# Autodesk Inventor assembly: SPE1V1 Estructura
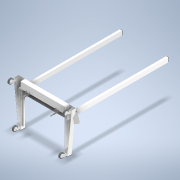
[picture p0: Inventor's stored thumbnail of the model, 180x180]
Saved by Autodesk Inventor 2021.2 (Build 252289000, 289)
## iProperties
Created: 2026-06-02
Part Number: SPE1V1 Estructura
Document SubType Name: Assembly
Designer: nelso
Author: nelso
## Documents named in this file (18)
- C:\Users\nelso\Desktop\Soporte-Paciente-Espinografia\Workspace\SPE1V1 Estructura.iam
- C:\Users\nelso\Desktop\Soporte-Paciente-Espinografia\Workspace\SP22V1 Tubo 40x80x1825mm.ipt
- C:\Users\nelso\Desktop\Soporte-Paciente-Espinografia\Workspace\SP21V1 Tubo 40x80x100mm.ipt
- C:\Users\nelso\Desktop\Soporte-Paciente-Espinografia\Workspace\SP23V1 Cobertora Derecha.ipt
- C:\Users\nelso\Desktop\Soporte-Paciente-Espinografia\Workspace\SP24V1 Cobertora Izquierda.ipt
- C:\Users\nelso\Desktop\Soporte-Paciente-Espinografia\Workspace\SP20V1 Tubo 80x120x790mm.ipt
- C:\Users\nelso\Desktop\Soporte-Paciente-Espinografia\Workspace\SP19V1 Tapacanto Delantero.ipt
- C:\Users\nelso\Desktop\Soporte-Paciente-Espinografia\Workspace\SP18V1 Tapacanto Superior.ipt
- C:\Users\nelso\Desktop\Soporte-Paciente-Espinografia\Workspace\RFPLUS8PO300.ipt
- C:\Users\nelso\Desktop\Soporte-Paciente-Espinografia\Workspace\SP17V1 Varilla Pedal.ipt
- C:\Users\nelso\Desktop\Soporte-Paciente-Espinografia\Workspace\SP16V1 Buje Pedal.ipt
- C:\Users\nelso\Desktop\Soporte-Paciente-Espinografia\Workspace\SP15V1 Pedal Izquierdo.ipt
- C:\Users\nelso\Desktop\Soporte-Paciente-Espinografia\Workspace\SPE3V1 Freno.iam
- C:\Users\nelso\Desktop\Soporte-Paciente-Espinografia\Workspace\SP14V1 Pedal Derecho.ipt
- C:\Users\nelso\Desktop\Soporte-Paciente-Espinografia\Workspace\5100B-HG-RU.ipt
- C:\Users\nelso\Desktop\Soporte-Paciente-Espinografia\Workspace\SP33V1 Tope Base.ipt
- C:\Users\nelso\Desktop\Soporte-Paciente-Espinografia\Workspace\SP38V1 Cobertor Freno.ipt
- C:\Users\nelso\Desktop\Soporte-Paciente-Espinografia\Workspace\SP43V1 Tubo 40x80x1825mm.ipt
## Components (42 placed, 17 different names)
1. SP43V1 Tubo 40x80x1825mm:1 — Nivelación:17, Coincidencia:54, Coincidencia:55, Coincidencia:68, Nivelación:67, Coincidencia:71, Flush:75, Flush:76, Flush:77, Flush:78, Flush:79, Mate:84, Mate:85, Mate:86, Mate:87, Mate:88, Mate:107, Flush:101
2. SP18V1 Tapacanto Superior:1 — Coincidencia:68, Nivelación:67, Coincidencia:71
3. SP22V1 Tubo 40x80x1825mm:2 — Mate:179, Mate:180, Flush:120, Mate:181, Mate:182, Mate:183, Mate:184, Mate:185, Mate:186, Mate:187, Flush:121, Flush:122, Flush:123, Flush:124, Flush:125, Flush:126
4. SP18V1 Tapacanto Superior:2 — Mate:181
5. SP21V1 Tubo 40x80x100mm:1 — Nivelación:14, Coincidencia:24, Coincidencia:42, Coincidencia:60, Coincidencia:62, Coincidencia:63, Mate:156, Mate:157
6. SP19V1 Tapacanto Delantero:1 — Coincidencia:60, Coincidencia:62, Coincidencia:63
7. SP21V1 Tubo 40x80x100mm:2 — Coincidencia:37, Coincidencia:38, Coincidencia:66, Mate:154, Mate:155
8. SP21V1 Tubo 40x80x100mm:3 — Coincidencia:50, Coincidencia:51, Coincidencia:65, Mate:158, Mate:159
9. SP21V1 Tubo 40x80x100mm:4 — Mate:150, Mate:151, Mate:160, Mate:161
10. SP19V1 Tapacanto Delantero:2 — Mate:152
11. SP23V1 Cobertora Derecha:1 — Nivelación:14, Coincidencia:24, Nivelación:17, Coincidencia:37, Coincidencia:38, Nivelación:18, Coincidencia:42, Nivelación:26, Coincidencia:55, Nivelación:27, Coincidencia:66, Flush:97, Flush:98, Mate:96, Mate:97, Flush:105, Mate:126, Mate:131, Mate:162, Mate:174, Flush:118
12. SP24V1 Cobertora Izquierda:1 — Nivelación:18, Coincidencia:50, Coincidencia:51, Nivelación:24, Coincidencia:53, Nivelación:28, Coincidencia:65, Flush:95, Flush:96, Mate:94, Mate:95, Flush:104, Mate:127, Mate:150, Mate:151, Mate:152, Mate:180, Flush:120
13. SP20V1 Tubo 80x120x790mm:1 — Nivelación:24, Nivelación:25, Coincidencia:54, Nivelación:27, Nivelación:28, Mate:110, Mate:111, Mate:124, Flush:119, Mate:177, Mate:179
14. RFPLUS8PO300:1 — Mate:107, Flush:101
15. RFPLUS8PO300:2 — Flush:75, Mate:88
16. RFPLUS8PO300:3 — Flush:76, Mate:87
17. RFPLUS8PO300:4 — Flush:77, Mate:86
18. RFPLUS8PO300:5 — Flush:78, Mate:84
19. RFPLUS8PO300:6 — Flush:79, Mate:85
20. RFPLUS8PO300:13 — Flush:95, Mate:94
21. RFPLUS8PO300:14 — Flush:96, Mate:95
22. RFPLUS8PO300:15 — Flush:97, Mate:97
23. RFPLUS8PO300:16 — Flush:98, Mate:96
24. SP17V1 Varilla Pedal:1 — Flush:102, Mate:117, Mate:118, Mate:119, Mate:120, Mate:121, Mate:125, Mate:128, Mate:129, Mate:130, Mate:132, Mate:133, Mate:134, Flush:106, Flush:107
25. SP16V1 Buje Pedal:1 — Mate:116, Flush:105, Mate:131
26. SP16V1 Buje Pedal:2 — Mate:116, Mate:125, Flush:104
27. SP14V1 Pedal Derecho:1 — Mate:128, Mate:129, Mate:130, Mate:132, Flush:107
28. SP15V1 Pedal Izquierdo:1 — Mate:120, Mate:121, Flush:106
29. SPE3V1 Freno:1 [sub-assembly] — Mate:110, Flush:103, Mate:117, Mate:118, Mate:119, Mate:124, Mate:127
30. SPE3V1 Freno:2 [sub-assembly] — Mate:111, Flush:103, Mate:126, Mate:133, Mate:134
31. RFPLUS8PO300:17 — Mate:187, Flush:121
32. RFPLUS8PO300:18 — Mate:186, Flush:122
33. RFPLUS8PO300:19 — Mate:185, Flush:123
34. RFPLUS8PO300:20 — Mate:184, Flush:124
35. RFPLUS8PO300:21 — Mate:182, Flush:125
36. RFPLUS8PO300:22 — Mate:183, Flush:126
37. 5100B-HG-RU:1 — Mate:154, Mate:155, Tangent:1
38. 5100B-HG-RU:2 — Mate:156, Mate:157
39. 5100B-HG-RU:3 — Mate:160, Mate:161
40. 5100B-HG-RU:4 — Mate:158, Mate:159
41. SP33V1 Tope Base:1 — Mate:174, Flush:118, Mate:178
42. SP38V1 Cobertor Freno:1 — Mate:176, Flush:119, Mate:177, Mate:178
## Relationships (110: Mate 74, Flush 35, Tangent 1)
- Nivelación:14 [Flush]: SP21V1 Tubo 40x80x100mm:1 ↔ SP23V1 Cobertora Derecha:1
- Coincidencia:24 [Mate] (0.5 mm): SP21V1 Tubo 40x80x100mm:1 ↔ SP23V1 Cobertora Derecha:1
- Nivelación:17 [Flush]: SP43V1 Tubo 40x80x1825mm:1 ↔ SP23V1 Cobertora Derecha:1
- Coincidencia:37 [Mate]: SP21V1 Tubo 40x80x100mm:2 ↔ SP23V1 Cobertora Derecha:1
- Coincidencia:38 [Mate]: SP21V1 Tubo 40x80x100mm:2 ↔ SP23V1 Cobertora Derecha:1
- Nivelación:18 [Flush]: SP23V1 Cobertora Derecha:1 ↔ SP24V1 Cobertora Izquierda:1
- Coincidencia:42 [Mate]: SP21V1 Tubo 40x80x100mm:1 ↔ SP23V1 Cobertora Derecha:1
- Coincidencia:50 [Mate]: SP21V1 Tubo 40x80x100mm:3 ↔ SP24V1 Cobertora Izquierda:1
- Coincidencia:51 [Mate]: SP21V1 Tubo 40x80x100mm:3 ↔ SP24V1 Cobertora Izquierda:1
- Nivelación:24 [Flush]: SP24V1 Cobertora Izquierda:1 ↔ SP20V1 Tubo 80x120x790mm:1
- Nivelación:25 [Flush]: SP20V1 Tubo 80x120x790mm:1
- Coincidencia:53 [Mate] (395 mm): SP24V1 Cobertora Izquierda:1
- Nivelación:26 [Flush] (395 mm): SP23V1 Cobertora Derecha:1
- Coincidencia:54 [Mate]: SP43V1 Tubo 40x80x1825mm:1 ↔ SP20V1 Tubo 80x120x790mm:1
- Coincidencia:55 [Mate]: SP43V1 Tubo 40x80x1825mm:1 ↔ SP23V1 Cobertora Derecha:1
- Nivelación:27 [Flush]: SP23V1 Cobertora Derecha:1 ↔ SP20V1 Tubo 80x120x790mm:1
- Nivelación:28 [Flush]: SP24V1 Cobertora Izquierda:1 ↔ SP20V1 Tubo 80x120x790mm:1
- Coincidencia:60 [Mate]: SP21V1 Tubo 40x80x100mm:1 ↔ SP19V1 Tapacanto Delantero:1
- Coincidencia:62 [Mate]: SP21V1 Tubo 40x80x100mm:1 ↔ SP19V1 Tapacanto Delantero:1
- Coincidencia:63 [Mate]: SP21V1 Tubo 40x80x100mm:1 ↔ SP19V1 Tapacanto Delantero:1
- Coincidencia:65 [Mate]: SP21V1 Tubo 40x80x100mm:3 ↔ SP24V1 Cobertora Izquierda:1
- Coincidencia:66 [Mate]: SP21V1 Tubo 40x80x100mm:2 ↔ SP23V1 Cobertora Derecha:1
- Coincidencia:68 [Mate]: SP43V1 Tubo 40x80x1825mm:1 ↔ SP18V1 Tapacanto Superior:1
- Nivelación:67 [Flush]: SP43V1 Tubo 40x80x1825mm:1 ↔ SP18V1 Tapacanto Superior:1
- Coincidencia:71 [Mate]: SP43V1 Tubo 40x80x1825mm:1 ↔ SP18V1 Tapacanto Superior:1
- Flush:75: SP43V1 Tubo 40x80x1825mm:1 ↔ RFPLUS8PO300:2
- Flush:76: SP43V1 Tubo 40x80x1825mm:1 ↔ RFPLUS8PO300:3
- Flush:77: SP43V1 Tubo 40x80x1825mm:1 ↔ RFPLUS8PO300:4
- Flush:78: SP43V1 Tubo 40x80x1825mm:1 ↔ RFPLUS8PO300:5
- Flush:79: SP43V1 Tubo 40x80x1825mm:1 ↔ RFPLUS8PO300:6
- Mate:84: SP43V1 Tubo 40x80x1825mm:1 ↔ RFPLUS8PO300:5
- Mate:85: SP43V1 Tubo 40x80x1825mm:1 ↔ RFPLUS8PO300:6
- Mate:86: SP43V1 Tubo 40x80x1825mm:1 ↔ RFPLUS8PO300:4
- Mate:87: SP43V1 Tubo 40x80x1825mm:1 ↔ RFPLUS8PO300:3
- Mate:88: SP43V1 Tubo 40x80x1825mm:1 ↔ RFPLUS8PO300:2
- Flush:95: SP24V1 Cobertora Izquierda:1 ↔ RFPLUS8PO300:13
- Flush:96: SP24V1 Cobertora Izquierda:1 ↔ RFPLUS8PO300:14
- Mate:94: SP24V1 Cobertora Izquierda:1 ↔ RFPLUS8PO300:13
- Mate:95: SP24V1 Cobertora Izquierda:1 ↔ RFPLUS8PO300:14
- Flush:97: SP23V1 Cobertora Derecha:1 ↔ RFPLUS8PO300:15
- Flush:98: SP23V1 Cobertora Derecha:1 ↔ RFPLUS8PO300:16
- Mate:96: SP23V1 Cobertora Derecha:1 ↔ RFPLUS8PO300:16
- Mate:97: SP23V1 Cobertora Derecha:1 ↔ RFPLUS8PO300:15
- Mate:107: SP43V1 Tubo 40x80x1825mm:1 ↔ RFPLUS8PO300:1
- Flush:101: SP43V1 Tubo 40x80x1825mm:1 ↔ RFPLUS8PO300:1
- Flush:102: SP17V1 Varilla Pedal:1
- Mate:110: SP20V1 Tubo 80x120x790mm:1 ↔ SPE3V1 Freno:1
- Mate:111: SP20V1 Tubo 80x120x790mm:1 ↔ SPE3V1 Freno:2
- Mate:116: SP16V1 Buje Pedal:1 ↔ SP16V1 Buje Pedal:2
- Flush:103: SPE3V1 Freno:1 ↔ SPE3V1 Freno:2
- Mate:117: SP17V1 Varilla Pedal:1 ↔ SPE3V1 Freno:1
- Mate:118: SP17V1 Varilla Pedal:1 ↔ SPE3V1 Freno:1
- Mate:119: SP17V1 Varilla Pedal:1 ↔ SPE3V1 Freno:1
- Mate:120: SP17V1 Varilla Pedal:1 ↔ SP15V1 Pedal Izquierdo:1
- Mate:121: SP17V1 Varilla Pedal:1 ↔ SP15V1 Pedal Izquierdo:1
- Mate:124: SP20V1 Tubo 80x120x790mm:1 ↔ SPE3V1 Freno:1
- Mate:125: SP17V1 Varilla Pedal:1 ↔ SP16V1 Buje Pedal:2
- Flush:104: SP24V1 Cobertora Izquierda:1 ↔ SP16V1 Buje Pedal:2
- Flush:105: SP23V1 Cobertora Derecha:1 ↔ SP16V1 Buje Pedal:1
- Mate:126 (100 mm): SP23V1 Cobertora Derecha:1 ↔ SPE3V1 Freno:2
- Mate:127 (100 mm): SP24V1 Cobertora Izquierda:1 ↔ SPE3V1 Freno:1
- Mate:128: SP17V1 Varilla Pedal:1 ↔ SP14V1 Pedal Derecho:1
- Mate:129: SP17V1 Varilla Pedal:1 ↔ SP14V1 Pedal Derecho:1
- Mate:130: SP17V1 Varilla Pedal:1 ↔ SP14V1 Pedal Derecho:1
- Mate:131: SP23V1 Cobertora Derecha:1 ↔ SP16V1 Buje Pedal:1
- Mate:132: SP17V1 Varilla Pedal:1 ↔ SP14V1 Pedal Derecho:1
- Mate:133: SP17V1 Varilla Pedal:1 ↔ SPE3V1 Freno:2
- Mate:134: SP17V1 Varilla Pedal:1 ↔ SPE3V1 Freno:2
- Flush:106: SP17V1 Varilla Pedal:1 ↔ SP15V1 Pedal Izquierdo:1
- Flush:107: SP17V1 Varilla Pedal:1 ↔ SP14V1 Pedal Derecho:1
- [Flush]: SP22V1 Tubo 40x80x1825mm:2 ↔ SP18V1 Tapacanto Superior:2
- [Mate]: SP22V1 Tubo 40x80x1825mm:2 ↔ SP18V1 Tapacanto Superior:2
- [Mate]: SP21V1 Tubo 40x80x100mm:4 ↔ SP19V1 Tapacanto Delantero:2
- [Mate]: SP21V1 Tubo 40x80x100mm:4 ↔ SP19V1 Tapacanto Delantero:2
- [Mate]: SP21V1 Tubo 40x80x100mm:4 ↔ SP19V1 Tapacanto Delantero:2
- Mate:150 (0.5 mm): SP21V1 Tubo 40x80x100mm:4 ↔ SP24V1 Cobertora Izquierda:1
- Mate:151: SP21V1 Tubo 40x80x100mm:4 ↔ SP24V1 Cobertora Izquierda:1
- Mate:152: SP19V1 Tapacanto Delantero:2 ↔ SP24V1 Cobertora Izquierda:1
- Mate:154: SP21V1 Tubo 40x80x100mm:2 ↔ 5100B-HG-RU:1
- Mate:155: SP21V1 Tubo 40x80x100mm:2 ↔ 5100B-HG-RU:1
- Mate:156: SP21V1 Tubo 40x80x100mm:1 ↔ 5100B-HG-RU:2
- Mate:157: SP21V1 Tubo 40x80x100mm:1 ↔ 5100B-HG-RU:2
- Mate:158: SP21V1 Tubo 40x80x100mm:3 ↔ 5100B-HG-RU:4
- Mate:159: SP21V1 Tubo 40x80x100mm:3 ↔ 5100B-HG-RU:4
- Mate:160: SP21V1 Tubo 40x80x100mm:4 ↔ 5100B-HG-RU:3
- Mate:161: SP21V1 Tubo 40x80x100mm:4 ↔ 5100B-HG-RU:3
- Mate:162: SP23V1 Cobertora Derecha:1
- Mate:174: SP23V1 Cobertora Derecha:1 ↔ SP33V1 Tope Base:1
- Flush:118: SP23V1 Cobertora Derecha:1 ↔ SP33V1 Tope Base:1
- Mate:176: SP38V1 Cobertor Freno:1
- Flush:119: SP20V1 Tubo 80x120x790mm:1 ↔ SP38V1 Cobertor Freno:1
- Mate:177: SP20V1 Tubo 80x120x790mm:1 ↔ SP38V1 Cobertor Freno:1
- Mate:178: SP33V1 Tope Base:1 ↔ SP38V1 Cobertor Freno:1
- Mate:179: SP22V1 Tubo 40x80x1825mm:2 ↔ SP20V1 Tubo 80x120x790mm:1
- Mate:180: SP22V1 Tubo 40x80x1825mm:2 ↔ SP24V1 Cobertora Izquierda:1
- Flush:120: SP22V1 Tubo 40x80x1825mm:2 ↔ SP24V1 Cobertora Izquierda:1
- Mate:181: SP22V1 Tubo 40x80x1825mm:2 ↔ SP18V1 Tapacanto Superior:2
- Mate:182: SP22V1 Tubo 40x80x1825mm:2 ↔ RFPLUS8PO300:21
- Mate:183: SP22V1 Tubo 40x80x1825mm:2 ↔ RFPLUS8PO300:22
- Mate:184: SP22V1 Tubo 40x80x1825mm:2 ↔ RFPLUS8PO300:20
- Mate:185: SP22V1 Tubo 40x80x1825mm:2 ↔ RFPLUS8PO300:19
- Mate:186: SP22V1 Tubo 40x80x1825mm:2 ↔ RFPLUS8PO300:18
- Mate:187: SP22V1 Tubo 40x80x1825mm:2 ↔ RFPLUS8PO300:17
- Flush:121: SP22V1 Tubo 40x80x1825mm:2 ↔ RFPLUS8PO300:17
- Flush:122: SP22V1 Tubo 40x80x1825mm:2 ↔ RFPLUS8PO300:18
- Flush:123: SP22V1 Tubo 40x80x1825mm:2 ↔ RFPLUS8PO300:19
- Flush:124: SP22V1 Tubo 40x80x1825mm:2 ↔ RFPLUS8PO300:20
- Flush:125: SP22V1 Tubo 40x80x1825mm:2 ↔ RFPLUS8PO300:21
- Flush:126: SP22V1 Tubo 40x80x1825mm:2 ↔ RFPLUS8PO300:22
- Tangent:1: 5100B-HG-RU:1
## Named parameters: d314_d103 = 0 mm, d315_d104 = 0 mm, d330_d90 = 0 mm, d331_d92 = 0 mm, d332_d93 = 0 mm
